# Autodesk Inventor assembly: ASY-PRS-DRS 940
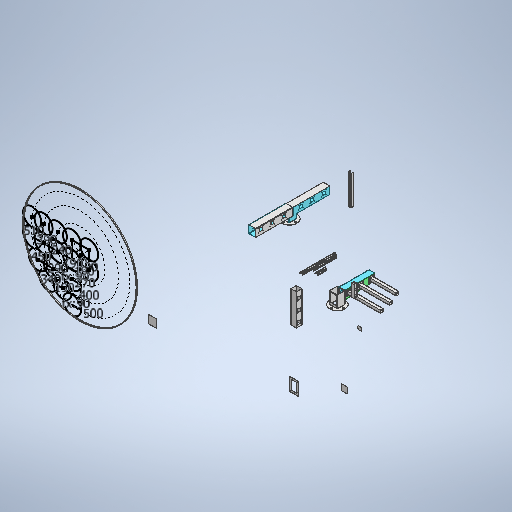
[picture p0: Inventor's stored thumbnail of the model, 512x512]
Saved by Autodesk Inventor 2026.2 (Build 302298000, 298)
## iProperties
Created: 2026-05-12
Part Number: ASY-PRS-DRS 940
Document SubType Name: Assembly
Designer: admin
Author: admin
## Documents named in this file (26)
- C:\Users\admin\Documents\Inventor\PRS-Purovsk\DRS 940\ASY-PRS-DRS 940.iam
- C:\Users\admin\Documents\Inventor\PRS-Purovsk\PRS-1425 FDS Way FLANGE.ipt
- C:\Users\admin\Documents\Inventor\PRS-Purovsk\ANP 1401 DSB DIMentions.ipt
- C:\Users\admin\Documents\Inventor\PRS-Purovsk\PRS-512 roof 2.ipt
- C:\Users\admin\Documents\Inventor\PRS-Purovsk\PRS-513 roof 3.ipt
- C:\Users\admin\Documents\Inventor\PRS-Purovsk\PRS-513 roof 4.ipt
- C:\Users\admin\Documents\Inventor\PRS-Purovsk\PRS-514 roof 4.ipt
- C:\Users\admin\Documents\Inventor\PRS-Purovsk\PRS-1661 (fds) main way tube.ipt
- C:\Users\admin\Documents\Inventor\PRS-Purovsk\PRS-1662 FDS 1000 way tube 4.ipt
- C:\Users\admin\Documents\Inventor\PRS-Purovsk\PRS-1651 FDS MAIN  FLANGE.ipt
- C:\Users\admin\Documents\Inventor\PRS-Purovsk\PRS-1652 FDS Central tube wall.ipt
- C:\Users\admin\Documents\Inventor\PRS-Purovsk\PRS-1661 FDS 1000 way tube 1.ipt
- C:\Users\admin\Documents\Inventor\PRS-Purovsk\PRS-1662 FDS 1000 way tube 2.ipt
- C:\Users\admin\Documents\Inventor\PRS-Purovsk\PRS-1663 FDS 1200 way tube 3.ipt
- C:\Users\admin\Documents\Inventor\PRS-Purovsk\PRS-1665 FDS 1000 CUP 1.ipt
- C:\Users\admin\Documents\Inventor\PRS-Purovsk\PRS-1666 FDS 1000 CUP 1.ipt
- C:\Users\admin\Documents\Inventor\PRS-Purovsk\PRS-1699 DIM filter-distribution-system 1000.ipt
- C:\Users\admin\Documents\Inventor\PRS-Purovsk\PRS-169859 DIM filter-distribution-system 1000.ipt
- C:\Users\admin\Documents\Inventor\PRS-Purovsk\PRS-1421 FDS Diam way flange 1.ipt
- C:\Users\admin\Documents\Inventor\PRS-Purovsk\PRS-1422 BOTTOM FDS diameter way up.ipt
- C:\Users\admin\Documents\Inventor\PRS-Purovsk\PRS-1423 BOTTOM FDS diameter way down.ipt
- C:\Users\admin\Documents\Inventor\PRS-Purovsk\PRS-1424 FDS diam way cup.ipt
- C:\Users\admin\Documents\Inventor\PRS-Purovsk\PRS-1422 BOTTOM FDS diameter way up_CPY.ipt
- C:\Users\admin\Documents\Inventor\PRS-Purovsk\PRS-1423 BOTTOM FDS diameter way down_CPY.ipt
- C:\Users\admin\Documents\Inventor\PRS-Purovsk\PRS-1651 FDS MAIN  FLANGE_CPY.ipt
- C:\Users\admin\Documents\Inventor\PRS-Purovsk\PRS-531 roof 1.ipt
## Components (33 placed, 25 different names)
1. PRS-169859 DIM filter-distribution-system 1000.ipt:1 — Mate:1, Mate:2, Flush:1
2. PRS-1425 FDS Way FLANGE.ipt:1 — Rigid:4, Rigid:19
3. ANP 1401 DSB DIMentions.ipt:1
4. PRS-512 roof 2.ipt:1
5. PRS-513 roof 3.ipt:1
6. PRS-513 roof 4.ipt:1
7. PRS-514 roof 4.ipt:1
8. PRS-1661 (fds) main way tube.ipt:1
9. PRS-1662 FDS 1000 way tube 4.ipt:1 — Rigid:21
10. PRS-1651 FDS MAIN  FLANGE.ipt:1 — Mate:3
11. PRS-1652 FDS Central tube wall.ipt:1 — Rigid:12
12. PRS-1662 FDS 1000 way tube 2.ipt:1 — Rigid:20
13. PRS-1663 FDS 1200 way tube 3.ipt:1
14. PRS-1665 FDS 1000 CUP 1.ipt:1
15. PRS-1666 FDS 1000 CUP 1.ipt:1
16. PRS-1699 DIM filter-distribution-system 1000.ipt:1
17. PRS-1421 FDS Diam way flange 1.ipt:1
18. PRS-1422 BOTTOM FDS diameter way up.ipt:1 — Rigid:13, Rigid:16, Rigid:17, Rigid:18
19. PRS-1423 BOTTOM FDS diameter way down.ipt:1 — Rigid:4, Rigid:12, Rigid:13, Rigid:14, Rigid:15
20. PRS-1424 FDS diam way cup.ipt:1
21. PRS-1652 FDS Central tube wall.ipt:2 — Mate:3
22. PRS-1422 BOTTOM FDS diameter way up_CPY.ipt:1 — Rigid:8
23. PRS-1423 BOTTOM FDS diameter way down_CPY.ipt:1 — Rigid:8
24. PRS-1423 BOTTOM FDS diameter way down_CPY.ipt:2 — Rigid:9
25. PRS-1422 BOTTOM FDS diameter way up_CPY.ipt:2 — Rigid:9
26. PRS-1651 FDS MAIN  FLANGE_CPY.ipt:1
27. PRS-1425 FDS Way FLANGE.ipt:2 — Rigid:14, Rigid:20
28. PRS-1425 FDS Way FLANGE.ipt:3 — Rigid:15, Rigid:21
29. PRS-1425 FDS Way FLANGE.ipt:4 — Rigid:18
30. PRS-1425 FDS Way FLANGE.ipt:5 — Rigid:17
31. PRS-1425 FDS Way FLANGE.ipt:6 — Rigid:16
32. PRS-1661 FDS 1000 way tube 1.ipt:1 — Rigid:19
33. PRS-531 roof 1:1
## Relationships (17: WeldJoint 13, Mate 3, Flush 1)
- Mate:1: PRS-169859 DIM filter-distribution-system 1000.ipt:1
- Mate:2: PRS-169859 DIM filter-distribution-system 1000.ipt:1
- Flush:1: PRS-169859 DIM filter-distribution-system 1000.ipt:1
- Rigid:4 [WeldJoint]: PRS-1425 FDS Way FLANGE.ipt:1 ↔ PRS-1423 BOTTOM FDS diameter way down.ipt:1
- Mate:3: PRS-1651 FDS MAIN  FLANGE.ipt:1 ↔ PRS-1652 FDS Central tube wall.ipt:2
- Rigid:8 [WeldJoint]: PRS-1422 BOTTOM FDS diameter way up_CPY.ipt:1 ↔ PRS-1423 BOTTOM FDS diameter way down_CPY.ipt:1
- Rigid:9 [WeldJoint]: PRS-1423 BOTTOM FDS diameter way down_CPY.ipt:2 ↔ PRS-1422 BOTTOM FDS diameter way up_CPY.ipt:2
- Rigid:12 [WeldJoint]: PRS-1652 FDS Central tube wall.ipt:1 ↔ PRS-1423 BOTTOM FDS diameter way down.ipt:1
- Rigid:13 [WeldJoint]: PRS-1422 BOTTOM FDS diameter way up.ipt:1 ↔ PRS-1423 BOTTOM FDS diameter way down.ipt:1
- Rigid:14 [WeldJoint]: PRS-1423 BOTTOM FDS diameter way down.ipt:1 ↔ PRS-1425 FDS Way FLANGE.ipt:2
- Rigid:15 [WeldJoint]: PRS-1423 BOTTOM FDS diameter way down.ipt:1 ↔ PRS-1425 FDS Way FLANGE.ipt:3
- Rigid:16 [WeldJoint]: PRS-1422 BOTTOM FDS diameter way up.ipt:1 ↔ PRS-1425 FDS Way FLANGE.ipt:6
- Rigid:17 [WeldJoint]: PRS-1422 BOTTOM FDS diameter way up.ipt:1 ↔ PRS-1425 FDS Way FLANGE.ipt:5
- Rigid:18 [WeldJoint]: PRS-1422 BOTTOM FDS diameter way up.ipt:1 ↔ PRS-1425 FDS Way FLANGE.ipt:4
- Rigid:19 [WeldJoint] (-2 mm): PRS-1425 FDS Way FLANGE.ipt:1 ↔ PRS-1661 FDS 1000 way tube 1.ipt:1
- Rigid:20 [WeldJoint] (-2 mm): PRS-1662 FDS 1000 way tube 2.ipt:1 ↔ PRS-1425 FDS Way FLANGE.ipt:2
- Rigid:21 [WeldJoint] (-2 mm): PRS-1662 FDS 1000 way tube 4.ipt:1 ↔ PRS-1425 FDS Way FLANGE.ipt:3
